# Autodesk Inventor assembly: Assembly8
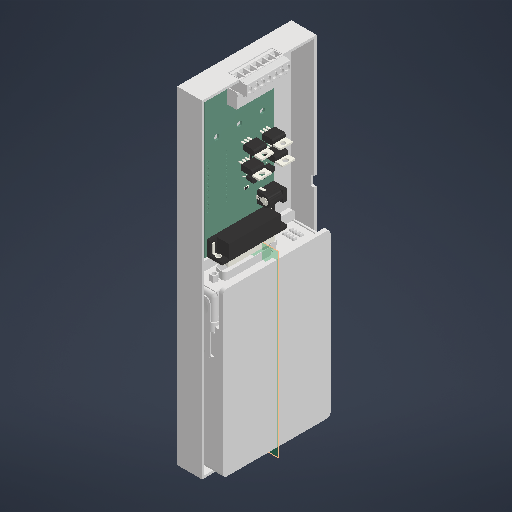
[picture p0: Inventor's stored thumbnail of the model, 512x512]
Saved by Autodesk Inventor 2027 (Build 310192000, 192)
## iProperties
Created: 2026-05-11
Part Number: Assembly8
Document SubType Name: Assembly
Designer: giese
Author: giese
## Documents named in this file (5)
- C:\Users\giese\OneDrive\Documents\GitHub\Biphasic-data-acquisition-system\DAQ_design\Assisi\v0.2.1\CAD\Assembly8.iam
- C:\Users\giese\OneDrive\Documents\Work\cdaq\cdaq.ipt
- C:\Users\giese\OneDrive\Documents\GitHub\Biphasic-data-acquisition-system\DAQ_design\Assisi\v0.2.1\EDA\assisi_v0.2.1\assisi_v0.2.1.ipt
- C:\Users\giese\OneDrive\Documents\GitHub\Biphasic-data-acquisition-system\DAQ_design\Assisi\v0.2.1\CAD\cDAQ_Bottom_Box3.ipt
- C:\Users\giese\OneDrive\Documents\GitHub\Biphasic-data-acquisition-system\DAQ_design\Assisi\v0.2.1\CAD\cDAQ_Chassis_LowPolyPlaceholder.ipt
## Components (4 placed, 4 different names)
1. cdaq:1 — Mate:3, Mate:4, Mate:5
2. assisi_v0.2.1:1 — Mate:6, Flush:1, Mate:7
3. cDAQ_Bottom_Box3:1 — Mate:1, Mate:2, Mate:6, Flush:1, Mate:7
4. cDAQ_Chassis_LowPolyPlaceholder:1 — Mate:1, Mate:2, Mate:3, Mate:4, Mate:5
## Relationships (8: Mate 7, Flush 1)
- Mate:1: cDAQ_Bottom_Box3:1 ↔ cDAQ_Chassis_LowPolyPlaceholder:1
- Mate:2: cDAQ_Bottom_Box3:1 ↔ cDAQ_Chassis_LowPolyPlaceholder:1
- Mate:3: cdaq:1 ↔ cDAQ_Chassis_LowPolyPlaceholder:1
- Mate:4: cdaq:1 ↔ cDAQ_Chassis_LowPolyPlaceholder:1
- Mate:5: cdaq:1 ↔ cDAQ_Chassis_LowPolyPlaceholder:1
- Mate:6: assisi_v0.2.1:1 ↔ cDAQ_Bottom_Box3:1
- Flush:1: assisi_v0.2.1:1 ↔ cDAQ_Bottom_Box3:1
- Mate:7: assisi_v0.2.1:1 ↔ cDAQ_Bottom_Box3:1
